# Autodesk Inventor assembly: brush holder assy v4
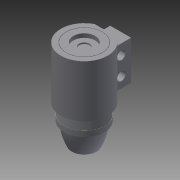
[picture p0: Inventor's stored thumbnail of the model, 180x180]
Saved by Autodesk Inventor 2013 SP2 (Build 170200200, 200)
## iProperties
Created: 2017-08-28
Part Number: brush holder assy v4
Document SubType Name: Assembly
Designer: hdv
Author: hdv
## Documents named in this file (5)
- C:\Users\Herman de Vries\Dropbox\Projects\Inventor\PaintBot_3\Brush holder\brush holder assy v4.iam
- C:\Users\Herman de Vries\Dropbox\Projects\Inventor\PaintBot_3\Brush holder\brush fitting partb.ipt
- C:\Users\Herman de Vries\Dropbox\Projects\Inventor\PaintBot_3\Brush holder\brush holder v4.ipt
- C:\Users\Herman de Vries\Dropbox\Projects\Inventor\PaintBot_3\Brush holder\brush fitting parta v4.ipt
- C:\Users\Herman de Vries\Dropbox\Projects\Inventor\PaintBot_3\Brush holder\magnet holder v4.ipt
## Components (4 placed, 4 different names)
1. brush holder v4:1 — Mate:5, Insert:1
2. brush fitting parta v4:1 — Mate:3, Mate:4, Mate:5
3. brush fitting partb:1 — Mate:3, Mate:4
4. magnet holder v4:1 — Insert:1
## Relationships (4: Mate 3, Insert 1)
- Mate:3: brush fitting parta v4:1 ↔ brush fitting partb:1
- Mate:4: brush fitting parta v4:1 ↔ brush fitting partb:1
- Mate:5: brush holder v4:1 ↔ brush fitting parta v4:1
- Insert:1: brush holder v4:1 ↔ magnet holder v4:1
